# Autodesk Inventor assembly: HeadBase
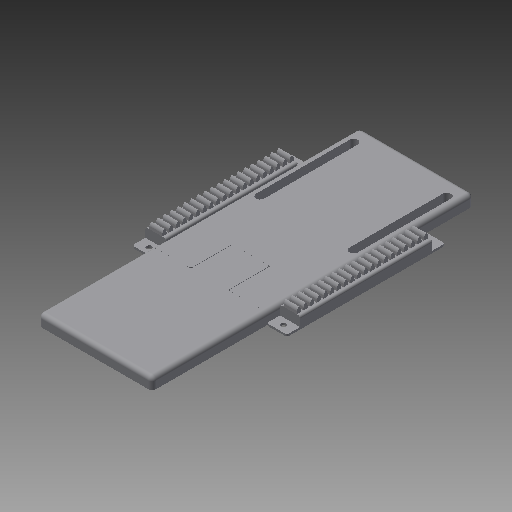
[picture p0: Inventor's stored thumbnail of the model, 512x512]
Saved by Autodesk Inventor 2018 (Build 220112000, 112)
## iProperties
Created: 2018-01-14
Part Number: HeadBase
Document SubType Name: Assembly
Designer: reide
Author: reide
## Documents named in this file (3)
- C:\Users\reide\OneDrive\Documents\Inventor\TSA\2018\Animatronics\Tortoise\Head\HeadBase.iam
- C:\Users\reide\OneDrive\Documents\Inventor\TSA\2018\Animatronics\Tortoise\Head\HeadBasePt1.iam
- C:\Users\reide\OneDrive\Documents\Inventor\TSA\2018\Animatronics\Tortoise\Head\HeadBasePt2.iam
## Components (2 placed, 2 different names)
1. HeadBasePt1:1 [sub-assembly] — Flush:1, Flush:2, Mate:1
2. HeadBasePt2:1 [sub-assembly] — Flush:1, Flush:2, Mate:1
## Relationships (3: Flush 2, Mate 1)
- Flush:1: HeadBasePt1:1 ↔ HeadBasePt2:1
- Flush:2: HeadBasePt1:1 ↔ HeadBasePt2:1
- Mate:1: HeadBasePt1:1 ↔ HeadBasePt2:1
